# Autodesk Inventor assembly: MP-42016-550
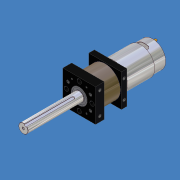
[picture p0: Inventor's stored thumbnail of the model, 180x180]
Saved by Autodesk Inventor 2015 (Build 190159000, 159)
## iProperties
Company: FirstCadLibrary
Shininess: 64.0
Length Units: 11272
Angle Units: 11279
Time Units: 11290
Mass Units: 11286
Length Display Precision: 3
Angle Display Precision: 2
Compacted: True
Part Number: MP-42016-550
Document SubType Name: Assembly
Created: 2007-01-14
Designer: Ed Sparks
Description: BaneBots 42mm Gearbox 16:1
Catalog Web Link: www.banebots.com
Vendor: BaneBots
Density: 0.0
Volumn: 0.0
Area: 0.0
PropertySet Name: Model Information
Control State: 0
Master: False
Checked Out: False
Title: BaneBots 42mm Gearbox 16:1
Author: Ed Sparks
## Documents named in this file (7)
- \\lhssvr02\Homedirs\Robotics Club\CAD Model 2015\Parts Folder\Gear Boxes\Bane Bots\16-1\BB-42016.iam
- \\lhssvr02\Homedirs\Robotics Club\CAD Model 2015\Parts Folder\Gear Boxes\Bane Bots\16-1\FisherPriceMotor.ipt
- \\lhssvr02\Homedirs\Robotics Club\CAD Model 2015\Parts Folder\Gear Boxes\Bane Bots\16-1\BB5-FrontPlate.ipt
- \\lhssvr02\Homedirs\Robotics Club\CAD Model 2015\Parts Folder\Gear Boxes\Bane Bots\16-1\BB5-Bearing.ipt
- \\lhssvr02\Homedirs\Robotics Club\CAD Model 2015\Parts Folder\Gear Boxes\Bane Bots\16-1\BB5-Axle.ipt
- \\lhssvr02\Homedirs\Robotics Club\CAD Model 2015\Parts Folder\Gear Boxes\Bane Bots\16-1\BB5-RingGear.ipt
- \\lhssvr02\Homedirs\Robotics Club\CAD Model 2015\Parts Folder\Gear Boxes\Bane Bots\16-1\BB5-BackPlate.ipt
## Components (7 placed, 6 different names)
1. BB5-FrontPlate:1 — Mate:3, Flush:1, Mate:6, Mate:7, Mate:8
2. BB5-Bearing:1 — Mate:1, Mate:2, Mate:3, Flush:1, Mate:4, Mate:5
3. BB5-Bearing:2 — Mate:1, Mate:2
4. BB5-Axle:1 — Mate:4, Mate:5
5. BB5-RingGear:1 — Mate:6, Mate:7, Mate:8, Mate:9, Mate:10, Mate:11
6. BB5-BackPlate:1 — Mate:9, Mate:10, Mate:11, Mate:12, Mate:13, Mate:14
7. FisherPriceMotor:1 — Mate:12, Mate:13, Mate:14
## Relationships (15: Mate 14, Flush 1)
- Mate:1: BB5-Bearing:1 ↔ BB5-Bearing:2
- Mate:2: BB5-Bearing:1 ↔ BB5-Bearing:2
- Mate:3: BB5-FrontPlate:1 ↔ BB5-Bearing:1
- Flush:1: BB5-FrontPlate:1 ↔ BB5-Bearing:1
- Mate:4: BB5-Bearing:1 ↔ BB5-Axle:1
- Mate:5: BB5-Bearing:1 ↔ BB5-Axle:1
- Mate:6: BB5-FrontPlate:1 ↔ BB5-RingGear:1
- Mate:7: BB5-FrontPlate:1 ↔ BB5-RingGear:1
- Mate:8: BB5-FrontPlate:1 ↔ BB5-RingGear:1
- Mate:9: BB5-RingGear:1 ↔ BB5-BackPlate:1
- Mate:10: BB5-RingGear:1 ↔ BB5-BackPlate:1
- Mate:11: BB5-RingGear:1 ↔ BB5-BackPlate:1
- Mate:12: BB5-BackPlate:1 ↔ FisherPriceMotor:1
- Mate:13: BB5-BackPlate:1 ↔ FisherPriceMotor:1
- Mate:14: BB5-BackPlate:1 ↔ FisherPriceMotor:1
